# Autodesk Inventor assembly: ASY GBK 1110 long wall shield 1_Dummy
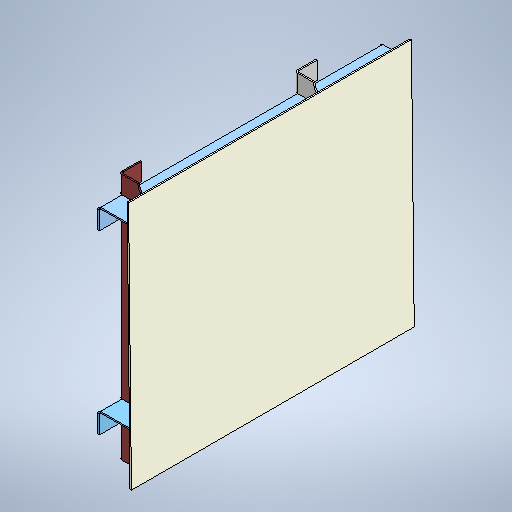
[picture p0: Inventor's stored thumbnail of the model, 512x512]
Saved by Autodesk Inventor 2026.2 (Build 302298010, 298A)
## iProperties
Created: 2026-05-07
Part Number: ASY GBK 1110 long wall shield 1_Dummy
Document SubType Name: Assembly
Designer: admin
Stock Number: 1111
Mass: 136093 g
Surface Area: 87957.2 cm^2
Volume: 17336.7 cm^3
Density: 7.85 g/cm^3
Author: admin
## Documents named in this file (5)
- C:\Users\admin\Desktop\GBK-Gubkinskiy\dummy\ASY GBK 1110 long wall shield 1_Dummy.iam
- C:\Users\admin\Desktop\GBK-Gubkinskiy\dummy\GBK 1111 shield 1_Dummy.ipt
- C:\Users\admin\Desktop\GBK-Gubkinskiy\dummy\GBK 0101 main rib_Dummy.ipt
- C:\Users\admin\Desktop\GBK-Gubkinskiy\dummy\GBK 0103 stringer 2_Dummy.ipt
- C:\Users\admin\Desktop\GBK-Gubkinskiy\dummy\GBK 0104 stringer 3_Dummy.ipt
## Components (5 placed, 4 different names)
1. GBK 1111 shield 1_Dummy:1 — Mate:1, Flush:1, Mate:6
2. GBK 0101 main rib_Dummy:1 — Mate:1, Rigid:1, Rigid:3, Mate:5
3. GBK 0103 stringer 2_Dummy:1 — Rigid:1, Rigid:2
4. GBK 0104 stringer 3_Dummy:1 — Rigid:3, Flush:1
5. GBK 0101 main rib_Dummy:2 — Rigid:2
## Relationships (7: Mate 3, WeldJoint 3, Flush 1)
- Mate:1: GBK 1111 shield 1_Dummy:1 ↔ GBK 0101 main rib_Dummy:1
- Rigid:1 [WeldJoint] (4 mm): GBK 0101 main rib_Dummy:1 ↔ GBK 0103 stringer 2_Dummy:1
- Rigid:2 [WeldJoint] (4 mm): GBK 0103 stringer 2_Dummy:1 ↔ GBK 0101 main rib_Dummy:2
- Rigid:3 [WeldJoint] (4 mm): GBK 0101 main rib_Dummy:1 ↔ GBK 0104 stringer 3_Dummy:1
- Mate:5: GBK 0101 main rib_Dummy:1
- Flush:1 (153 mm): GBK 1111 shield 1_Dummy:1 ↔ GBK 0104 stringer 3_Dummy:1
- Mate:6: GBK 1111 shield 1_Dummy:1
